# Autodesk Inventor assembly: front_panel_2004
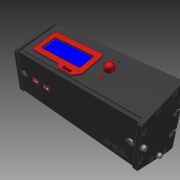
[picture p0: Inventor's stored thumbnail of the model, 180x180]
Saved by Autodesk Inventor 2014 (Build 180170000, 170)
## iProperties
Created: 2014-01-23
Part Number: front_panel_2004
Document SubType Name: Assembly
Designer: buben
Author: buben
## Documents named in this file (14)
- C:\Users\buben\Documents\GitHub\bacon\inventor files\assemblies\front_panel_2004.iam
- C:\Users\buben\Documents\GitHub\bacon\inventor files\printer parts\front_panel_2004_display.ipt
- C:\Users\buben\Documents\GitHub\bacon\inventor files\3rd party components\ramps 1.4 controller\Imported Components\lcd\lcd.ipt
- C:\Users\buben\Documents\GitHub\bacon\inventor files\printer parts\front_panel_2004_brace_right.ipt
- C:\Users\buben\Documents\GitHub\bacon\inventor files\utils\display_2004_frame.ipt
- C:\Users\buben\Documents\GitHub\bacon\inventor files\printer parts\front_panel_2004_front.ipt
- C:\Users\buben\Documents\GitHub\bacon\inventor files\printer parts\front_panel_2004_bottom.ipt
- C:\Users\buben\Documents\GitHub\bacon\inventor files\printer parts\front_panel_2004_brace_left.ipt
- C:\Users\buben\Documents\GitHub\bacon\inventor files\utils\washer_m4.ipt
- C:\Users\buben\Documents\Inventor\Content Center Files\R2014\en-US\ISO 4762(2)\ISO 4762 - M4 x 20ISO.ipt
- C:\Users\buben\Documents\Inventor\Content Center Files\R2014\en-US\ISO 7040\ISO 7040 - M4.ipt
- C:\Users\buben\Documents\GitHub\bacon\inventor files\3rd party components\USB socket\Imported Components\USB-Socket\USB-Socket.ipt
- C:\Users\buben\Documents\GitHub\bacon\inventor files\utils\controller_push_button.ipt
- C:\Users\buben\Documents\GitHub\bacon\inventor files\utils\rotary_encoder_cnob.ipt
## Components (27 placed, 13 different names)
1. front_panel_2004_display:1 — Flush:2, Mate:2, Mate:3, Mate:4, Mate:5, Flush:5, Mate:10, Mate:14, Mate:16, Mate:49
2. lcd:1 — Flush:2, Mate:2, Mate:3, Flush:3, Flush:4, Mate:47, Mate:48, Mate:50
3. display_2004_frame:1 — Mate:4, Flush:3, Flush:4
4. front_panel_2004_brace_right:1 — Mate:5, Flush:5, Mate:6, Mate:7, Mate:8, Flush:7, Mate:11, Mate:12, Mate:13, Mate:21, Mate:22, Mate:23, Mate:24
5. front_panel_2004_front:1 — Mate:6, Mate:7, Mate:8, Flush:6, Mate:9, Mate:10, Mate:15, Mate:25, Mate:29, Mate:41, Mate:42, Mate:43, Mate:44, Mate:45, Mate:46
6. front_panel_2004_bottom:1 — Mate:11, Mate:12, Mate:13, Mate:27, Mate:31
7. front_panel_2004_brace_left:1 — Mate:14, Mate:15, Mate:16, Mate:17, Mate:18, Mate:19, Mate:20
8. CSN 02 1702 B B 4,3:1 — Mate:29, Mate:30, Mate:37
9. CSN 02 1702 B B 4,3:2 — Mate:31, Mate:32, Mate:39
10. CSN 02 1702 B B 4,3:3 — Mate:25, Mate:26, Mate:33
11. CSN 02 1702 B B 4,3:4 — Mate:27, Mate:28, Mate:35
12. CSN 02 1702 B B 4,3:5 — Mate:23, Mate:24, Insert:2
13. CSN 02 1702 B B 4,3:6 — Mate:21, Mate:22, Insert:1
14. CSN 02 1702 B B 4,3:7 — Mate:17, Mate:20, Insert:3
15. CSN 02 1702 B B 4,3:8 — Mate:18, Mate:19, Insert:4
16. ISO 4762 M4 x 20:1 — Insert:4, Mate:32, Mate:40
17. ISO 4762 M4 x 20:2 — Insert:3, Mate:30, Mate:38
18. ISO 4762 M4 x 20:3 — Insert:2, Mate:28, Mate:36
19. ISO 4762 M4 x 20:4 — Insert:1, Mate:26, Mate:34
20. DIN EN ISO 7040 M4:1 — Mate:35, Mate:36
21. DIN EN ISO 7040 M4:2 — Mate:33, Mate:34
22. DIN EN ISO 7040 M4:3 — Mate:39, Mate:40
23. DIN EN ISO 7040 M4:4 — Mate:37, Mate:38
24. USB-Socket:1 — Mate:41, Mate:43, Mate:46
25. USB-Socket:2 — Mate:42, Mate:44, Mate:45
26. controller_push_button:1 — Mate:49, Mate:50
27. rotary_encoder_cnob:1 — Mate:47, Mate:48
## Relationships (59: Mate 49, Flush 6, Insert 4)
- Flush:2: front_panel_2004_display:1 ↔ lcd:1
- Mate:2: front_panel_2004_display:1 ↔ lcd:1
- Mate:3: front_panel_2004_display:1 ↔ lcd:1
- Mate:4: front_panel_2004_display:1 ↔ display_2004_frame:1
- Flush:3 (1 mm): lcd:1 ↔ display_2004_frame:1
- Flush:4 (-1 mm): lcd:1 ↔ display_2004_frame:1
- Mate:5: front_panel_2004_display:1 ↔ front_panel_2004_brace_right:1
- Flush:5 (3 mm): front_panel_2004_display:1 ↔ front_panel_2004_brace_right:1
- Mate:6: front_panel_2004_brace_right:1 ↔ front_panel_2004_front:1
- Mate:7: front_panel_2004_brace_right:1 ↔ front_panel_2004_front:1
- Mate:8: front_panel_2004_brace_right:1 ↔ front_panel_2004_front:1
- Flush:6: front_panel_2004_front:1
- Mate:9: front_panel_2004_front:1
- Flush:7: front_panel_2004_brace_right:1
- Mate:10 (1 mm): front_panel_2004_display:1 ↔ front_panel_2004_front:1
- Mate:11: front_panel_2004_brace_right:1 ↔ front_panel_2004_bottom:1
- Mate:12: front_panel_2004_brace_right:1 ↔ front_panel_2004_bottom:1
- Mate:13: front_panel_2004_brace_right:1 ↔ front_panel_2004_bottom:1
- Mate:14: front_panel_2004_display:1 ↔ front_panel_2004_brace_left:1
- Mate:15: front_panel_2004_front:1 ↔ front_panel_2004_brace_left:1
- Mate:16: front_panel_2004_display:1 ↔ front_panel_2004_brace_left:1
- Mate:17: front_panel_2004_brace_left:1 ↔ CSN 02 1702 B B 4,3:7
- Mate:18: front_panel_2004_brace_left:1 ↔ CSN 02 1702 B B 4,3:8
- Mate:19: front_panel_2004_brace_left:1 ↔ CSN 02 1702 B B 4,3:8
- Mate:20: front_panel_2004_brace_left:1 ↔ CSN 02 1702 B B 4,3:7
- Mate:21: front_panel_2004_brace_right:1 ↔ CSN 02 1702 B B 4,3:6
- Mate:22: front_panel_2004_brace_right:1 ↔ CSN 02 1702 B B 4,3:6
- Mate:23: front_panel_2004_brace_right:1 ↔ CSN 02 1702 B B 4,3:5
- Mate:24: front_panel_2004_brace_right:1 ↔ CSN 02 1702 B B 4,3:5
- Insert:1: CSN 02 1702 B B 4,3:6 ↔ ISO 4762 M4 x 20:4
- Insert:2: CSN 02 1702 B B 4,3:5 ↔ ISO 4762 M4 x 20:3
- Insert:3: CSN 02 1702 B B 4,3:7 ↔ ISO 4762 M4 x 20:2
- Insert:4: CSN 02 1702 B B 4,3:8 ↔ ISO 4762 M4 x 20:1
- Mate:25: front_panel_2004_front:1 ↔ CSN 02 1702 B B 4,3:3
- Mate:26: CSN 02 1702 B B 4,3:3 ↔ ISO 4762 M4 x 20:4
- Mate:27: front_panel_2004_bottom:1 ↔ CSN 02 1702 B B 4,3:4
- Mate:28: CSN 02 1702 B B 4,3:4 ↔ ISO 4762 M4 x 20:3
- Mate:29: front_panel_2004_front:1 ↔ CSN 02 1702 B B 4,3:1
- Mate:30: CSN 02 1702 B B 4,3:1 ↔ ISO 4762 M4 x 20:2
- Mate:31: front_panel_2004_bottom:1 ↔ CSN 02 1702 B B 4,3:2
- Mate:32: CSN 02 1702 B B 4,3:2 ↔ ISO 4762 M4 x 20:1
- Mate:33: CSN 02 1702 B B 4,3:3 ↔ DIN EN ISO 7040 M4:2
- Mate:34: ISO 4762 M4 x 20:4 ↔ DIN EN ISO 7040 M4:2
- Mate:35: CSN 02 1702 B B 4,3:4 ↔ DIN EN ISO 7040 M4:1
- Mate:36: ISO 4762 M4 x 20:3 ↔ DIN EN ISO 7040 M4:1
- Mate:37: CSN 02 1702 B B 4,3:1 ↔ DIN EN ISO 7040 M4:4
- Mate:38: ISO 4762 M4 x 20:2 ↔ DIN EN ISO 7040 M4:4
- Mate:39: CSN 02 1702 B B 4,3:2 ↔ DIN EN ISO 7040 M4:3
- Mate:40: ISO 4762 M4 x 20:1 ↔ DIN EN ISO 7040 M4:3
- Mate:41: front_panel_2004_front:1 ↔ USB-Socket:1
- Mate:42: front_panel_2004_front:1 ↔ USB-Socket:2
- Mate:43 (0.5 mm): front_panel_2004_front:1 ↔ USB-Socket:1
- Mate:44 (0.5 mm): front_panel_2004_front:1 ↔ USB-Socket:2
- Mate:45 (0.5 mm): front_panel_2004_front:1 ↔ USB-Socket:2
- Mate:46 (0.5 mm): front_panel_2004_front:1 ↔ USB-Socket:1
- Mate:47: lcd:1 ↔ rotary_encoder_cnob:1
- Mate:48: lcd:1 ↔ rotary_encoder_cnob:1
- Mate:49: front_panel_2004_display:1 ↔ controller_push_button:1
- Mate:50: lcd:1 ↔ controller_push_button:1
